# Autodesk Inventor assembly: end door assembly.ipt
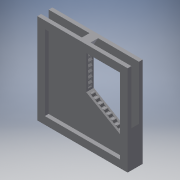
[picture p0: Inventor's stored thumbnail of the model, 180x180]
Saved by Autodesk Inventor 2017 (Build 210142000, 142)
## iProperties
Created: 2018-03-10
Part Number: end door assembly.ipt
Document SubType Name: Assembly
Designer: Braxton
Author: Braxton
## Documents named in this file (4)
- E:\School\Game develpment\geoscape\doors\end door\end door assembly.ipt.iam
- E:\School\Game develpment\geoscape\doors\end door\end door frame.ipt
- E:\School\Game develpment\geoscape\doors\end door\bottom door.ipt
- E:\School\Game develpment\geoscape\doors\end door\top left door.ipt
## Components (3 placed, 3 different names)
1. end door frame:1 — Mate:1, Mate:2, Mate:3, Mate:5
2. bottom door:1 — Mate:1, Mate:2, Mate:3, Mate:4, Mate:6
3. top left door:1 — Mate:4, Mate:5, Mate:6
## Relationships (6: Mate 6)
- Mate:1: end door frame:1 ↔ bottom door:1
- Mate:2: end door frame:1 ↔ bottom door:1
- Mate:3: end door frame:1 ↔ bottom door:1
- Mate:4: bottom door:1 ↔ top left door:1
- Mate:5: end door frame:1 ↔ top left door:1
- Mate:6: bottom door:1 ↔ top left door:1
